# Autodesk Inventor assembly: CameraUnit
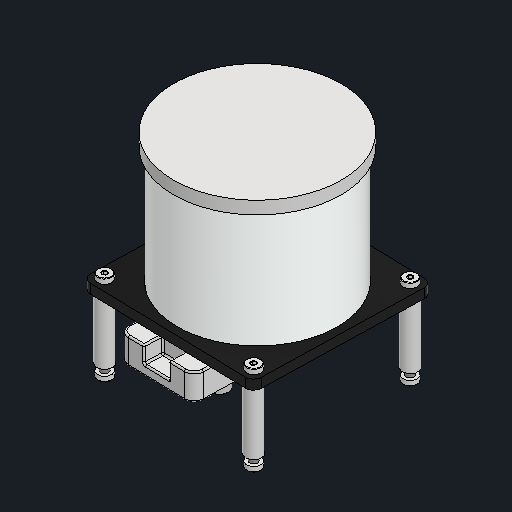
[picture p0: Inventor's stored thumbnail of the model, 512x512]
Saved by Autodesk Inventor 2024.2 (Build 282272000, 272)
## iProperties
Created: 2023-12-21
Part Number: CameraUnit
Document SubType Name: Assembly
Designer: Hanaoka
Author: Hanaoka
## Documents named in this file (8)
- G:\共有ドライブ\reRo\05_個人\hanaoka\inventor\CameraUnit\CameraUnit.iam
- G:\共有ドライブ\reRo\05_個人\hanaoka\inventor\CameraUnit\Camera_pipe.ipt
- G:\共有ドライブ\reRo\05_個人\hanaoka\inventor\Spacer\Spacer_M2.6x20.ipt
- G:\共有ドライブ\reRo\05_個人\hanaoka\inventor\Screw\M2.6x8\M2.6x8.ipt
- G:\共有ドライブ\reRo\05_個人\hanaoka\inventor\CameraUnit\UnitV_Mount.ipt
- G:\共有ドライブ\reRo\05_個人\hanaoka\inventor\CameraUnit\UnitV_OV7740_M12.ipt
- G:\共有ドライブ\reRo\05_個人\hanaoka\inventor\CameraUnit\cone_mirror.ipt
- G:\共有ドライブ\reRo\05_個人\hanaoka\inventor\Screw\M3x6.ipt
## Components (18 placed, 7 different names)
1. Camera_pipe:1 — 挿入:15, 挿入:16
2. Spacer_M2.6x20:1 — 挿入:2, 挿入:9
3. Spacer_M2.6x20:2 — 挿入:3, 挿入:10
4. Spacer_M2.6x20:3 — 挿入:4, 挿入:12
5. Spacer_M2.6x20:4 — 挿入:1, 挿入:11
6. M2.6x8:1 — 挿入:5
7. M2.6x8:2 — 挿入:6
8. M2.6x8:3 — 挿入:7
9. M2.6x8:4 — 挿入:8
10. M2.6x8:5 — 挿入:10
11. M2.6x8:6 — 挿入:9
12. M2.6x8:7 — 挿入:12
13. M2.6x8:8 — 挿入:11
14. UnitV_Mount:1 — 挿入:1, 挿入:2, 挿入:3, 挿入:4, 挿入:5, 挿入:6, 挿入:7, 挿入:8, 挿入:15, 挿入:19, 挿入:20
15. UnitV_OV7740_M12:1 — 挿入:17, 挿入:18, 挿入:19, 挿入:20
16. cone_mirror:1 — 挿入:16
17. M3x6:1 — 挿入:17
18. M3x6:2 — 挿入:18
## Relationships (18: Insert 18)
- 挿入:1 [Insert]: Spacer_M2.6x20:4 ↔ UnitV_Mount:1
- 挿入:2 [Insert]: Spacer_M2.6x20:1 ↔ UnitV_Mount:1
- 挿入:3 [Insert]: Spacer_M2.6x20:2 ↔ UnitV_Mount:1
- 挿入:4 [Insert]: Spacer_M2.6x20:3 ↔ UnitV_Mount:1
- 挿入:5 [Insert]: M2.6x8:1 ↔ UnitV_Mount:1
- 挿入:6 [Insert]: M2.6x8:2 ↔ UnitV_Mount:1
- 挿入:7 [Insert]: M2.6x8:3 ↔ UnitV_Mount:1
- 挿入:8 [Insert]: M2.6x8:4 ↔ UnitV_Mount:1
- 挿入:9 [Insert] (2 mm): Spacer_M2.6x20:1 ↔ M2.6x8:6
- 挿入:10 [Insert] (2 mm): Spacer_M2.6x20:2 ↔ M2.6x8:5
- 挿入:11 [Insert] (2 mm): Spacer_M2.6x20:4 ↔ M2.6x8:8
- 挿入:12 [Insert] (2 mm): Spacer_M2.6x20:3 ↔ M2.6x8:7
- 挿入:15 [Insert]: Camera_pipe:1 ↔ UnitV_Mount:1
- 挿入:16 [Insert]: Camera_pipe:1 ↔ cone_mirror:1
- 挿入:17 [Insert]: UnitV_OV7740_M12:1 ↔ M3x6:1
- 挿入:18 [Insert]: UnitV_OV7740_M12:1 ↔ M3x6:2
- 挿入:19 [Insert]: UnitV_Mount:1 ↔ UnitV_OV7740_M12:1
- 挿入:20 [Insert]: UnitV_Mount:1 ↔ UnitV_OV7740_M12:1
